# Autodesk Inventor assembly: Top
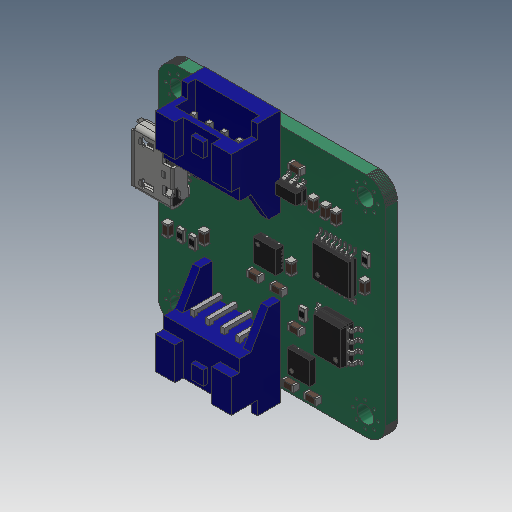
[picture p0: Inventor's stored thumbnail of the model, 512x512]
Saved by Autodesk Inventor 2019.4 (Build 234330000, 330)
## iProperties
Created: 2019-12-27
Part Number: Top
Material: 一般
Document SubType Name: Assembly
Designer: y6tada
Author: y6tada
## Documents named in this file (26)
- C:\Workspace\QUIKS\Hardware\IMUTracker\Circuit\IMUTracker_Inveotor_model\Top.iam
- C:\Workspace\QUIKS\Hardware\IMUTracker\Circuit\IMUTracker_Inveotor_model\C11_C_0603_5C47C8DF.ipt
- C:\Workspace\QUIKS\Hardware\IMUTracker\Circuit\IMUTracker_Inveotor_model\U2_TSSOP_16_44x5mm_Pitch065mm_5C47CB0E.ipt
- C:\Workspace\QUIKS\Hardware\IMUTracker\Circuit\IMUTracker_Inveotor_model\C1_C_0603_5C47C846.ipt
- C:\Workspace\QUIKS\Hardware\IMUTracker\Circuit\IMUTracker_Inveotor_model\C2_C_0603_5C47C857.ipt
- C:\Workspace\QUIKS\Hardware\IMUTracker\Circuit\IMUTracker_Inveotor_model\C3_C_0603_5C47C868.ipt
- C:\Workspace\QUIKS\Hardware\IMUTracker\Circuit\IMUTracker_Inveotor_model\C4_C_0603_5C47C879.ipt
- C:\Workspace\QUIKS\Hardware\IMUTracker\Circuit\IMUTracker_Inveotor_model\C6_C_0603_5C47C88A.ipt
- C:\Workspace\QUIKS\Hardware\IMUTracker\Circuit\IMUTracker_Inveotor_model\C7_C_0603_5C47C89B.ipt
- C:\Workspace\QUIKS\Hardware\IMUTracker\Circuit\IMUTracker_Inveotor_model\C8_C_0603_5C47C8AC.ipt
- C:\Workspace\QUIKS\Hardware\IMUTracker\Circuit\IMUTracker_Inveotor_model\C9_C_0603_5C47C8BD.ipt
- C:\Workspace\QUIKS\Hardware\IMUTracker\Circuit\IMUTracker_Inveotor_model\C10_C_0603_5C47C8CE.ipt
- C:\Workspace\QUIKS\Hardware\IMUTracker\Circuit\IMUTracker_Inveotor_model\C12_C_0603_5C47C8F0.ipt
- C:\Workspace\QUIKS\Hardware\IMUTracker\Circuit\IMUTracker_Inveotor_model\D1_C_0603_5C47C905.ipt
- C:\Workspace\QUIKS\Hardware\IMUTracker\Circuit\IMUTracker_Inveotor_model\R1_R_0603_5C47CAA6.ipt
- C:\Workspace\QUIKS\Hardware\IMUTracker\Circuit\IMUTracker_Inveotor_model\R2_R_0603_5C47CAB7.ipt
- C:\Workspace\QUIKS\Hardware\IMUTracker\Circuit\IMUTracker_Inveotor_model\R3_R_0603_5C47CAC8.ipt
- C:\Workspace\QUIKS\Hardware\IMUTracker\Circuit\IMUTracker_Inveotor_model\R4_R_0603_5C47CAD9.ipt
- C:\Workspace\QUIKS\Hardware\IMUTracker\Circuit\IMUTracker_Inveotor_model\U1_SOT_23_5_5C47CAEE.ipt
- C:\Workspace\QUIKS\Hardware\IMUTracker\Circuit\IMUTracker_Inveotor_model\U3_DFN-12-1EP_3x3mm_Pitch0.45mm_5C47CB2D.ipt
- C:\Workspace\QUIKS\Hardware\IMUTracker\Circuit\IMUTracker_Inveotor_model\U4_SOIC-8_3.9x4.9mm_Pitch1.27mm_5C47CB4A.ipt
- C:\Workspace\QUIKS\Hardware\IMUTracker\Circuit\IMUTracker_Inveotor_model\U5_QFN-24-1EP_3x3mm_Pitch0.4mm_5C47CB7A.ipt
- C:\Workspace\QUIKS\Hardware\IMUTracker\Circuit\IMUTracker_Inveotor_model\C5_C_0603_5C47D793.ipt
- C:\Workspace\QUIKS\Hardware\IMUTracker\Circuit\IMUTracker_Inveotor_model\J4_USB_Micro-B_Molex_47346-0001_5C544C86.ipt
- C:\Workspace\QUIKS\Hardware\IMUTracker\Circuit\IMUTracker_Inveotor_model\S04B-PASK-2.ipt
- C:\Workspace\QUIKS\Hardware\IMUTracker\Circuit\IMUTracker_Inveotor_model\Board_Geoms.iam
## Components (26 placed, 25 different names)
1. 33 [sub-assembly] — メイト:1, メイト:2, フラッシュ:2, フラッシュ:3, フラッシュ:4
2. 34
3. 35
4. 36
5. 37
6. 38
7. 39
8. 40
9. 41
10. 42
11. 43
12. 44
13. 45
14. 46
15. 47
16. 48
17. 49
18. 50
19. 51
20. 52
21. 53
22. 54
23. 55
24. 58
25. S04B-PASK-2:1 — メイト:1, フラッシュ:1, フラッシュ:2, フラッシュ:3
26. S04B-PASK-2:2 — メイト:2, フラッシュ:1, フラッシュ:4
## Relationships (6: Flush 4, Mate 2)
- メイト:1 [Mate]: 33 ↔ S04B-PASK-2:1
- メイト:2 [Mate]: 33 ↔ S04B-PASK-2:2
- フラッシュ:1 [Flush]: S04B-PASK-2:1 ↔ S04B-PASK-2:2
- フラッシュ:2 [Flush] (6.16 mm): 33 ↔ S04B-PASK-2:1
- フラッシュ:3 [Flush] (1.7 mm): 33 ↔ S04B-PASK-2:1
- フラッシュ:4 [Flush] (-1.7 mm): 33 ↔ S04B-PASK-2:2
